# Autodesk Inventor assembly: Beau4tClock
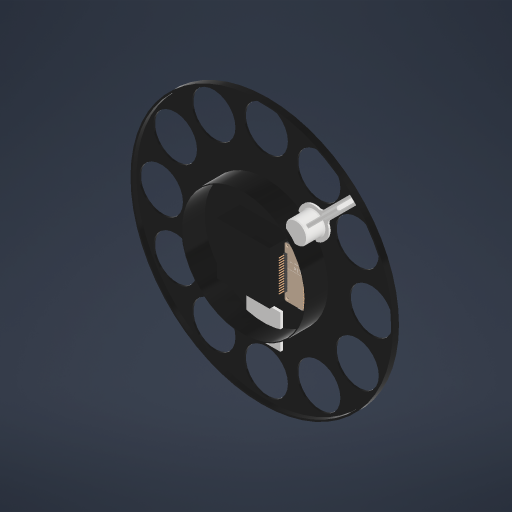
[picture p0: Inventor's stored thumbnail of the model, 512x512]
Saved by Autodesk Inventor 2023.1 (Build 271208000, 208)
## iProperties
Created: 2023-08-24
Part Number: Beau4tClock
Document SubType Name: Assembly
Designer: washichi
Author: washichi
## Documents named in this file (9)
- D:\Documents\Projects\WindForecastClock\3Dfiles\Beau4tClock.iam
- D:\Documents\Projects\WindForecastClock\3Dfiles\Clock.ipt
- D:\Documents\Projects\WindForecastClock\3Dfiles\LedStripV2.ipt
- D:\Documents\Projects\WindForecastClock\3Dfiles\HourGuard.ipt
- D:\Documents\Projects\WindForecastClock\3Dfiles\LedMatrix_WS2812_5x5.ipt
- D:\Documents\Projects\WindForecastClock\3Dfiles\Lolin NodeMCU ESP8266 V3.ipt
- D:\Documents\Projects\WindForecastClock\3Dfiles\LedStrip_36.ipt
- D:\Documents\Projects\WindForecastClock\3Dfiles\LedStrip_24.ipt
- D:\Documents\Projects\WindForecastClock\3Dfiles\HourGuard_36_wavyV2.ipt
## Components (8 placed, 8 different names)
1. Clock:1 — Flush:1, Flush:2, Flush:3, Flush:4, Flush:5, Flush:6, Flush:7, Flush:8, Flush:10, Flush:11, Flush:12
2. LedStrip_24:1 — Flush:10, Flush:11
3. LedStrip_30:1 — Flush:1, Flush:2
4. LedStrip_36:1 — Flush:7, Flush:8
5. HourGuard_30:1 — Flush:3, Flush:4
6. LedMatrix_WS2812_5x5:1 — Flush:5, Flush:6
7. Lolin NodeMCU ESP8266 V3:1
8. HourGuard_36_wavyV2:1 — Flush:12
## Relationships (11: Flush 11)
- Flush:1: Clock:1 ↔ LedStrip_30:1
- Flush:2 (2 mm): Clock:1 ↔ LedStrip_30:1
- Flush:3: Clock:1 ↔ HourGuard_30:1
- Flush:4: Clock:1 ↔ HourGuard_30:1
- Flush:5: Clock:1 ↔ LedMatrix_WS2812_5x5:1
- Flush:6: Clock:1 ↔ LedMatrix_WS2812_5x5:1
- Flush:7: Clock:1 ↔ LedStrip_36:1
- Flush:8 (5 mm): Clock:1 ↔ LedStrip_36:1
- Flush:10: Clock:1 ↔ LedStrip_24:1
- Flush:11 (5 mm): Clock:1 ↔ LedStrip_24:1
- Flush:12: Clock:1 ↔ HourGuard_36_wavyV2:1
